# Autodesk Inventor assembly: Electronics
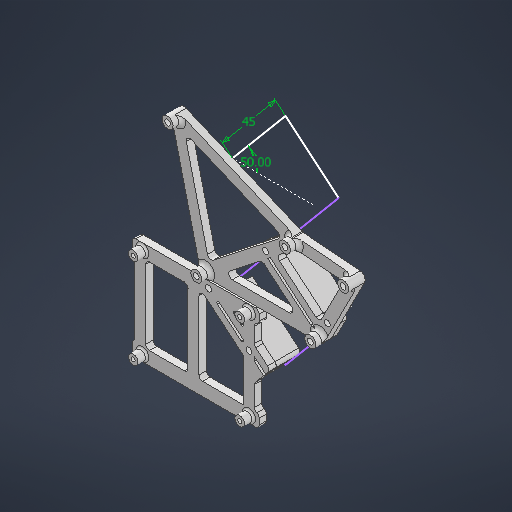
[picture p0: Inventor's stored thumbnail of the model, 512x512]
Saved by Autodesk Inventor 2025 (Build 290162000, 162)
## iProperties
Created: 2024-10-13
Part Number: Electronics
Document SubType Name: Assembly
Designer: Windows 7 was better
Author: Windows 7 was better
## Documents named in this file (6)
- C:\Users\Windows 7 was better\GitHub\ReplicatorPlusConversion\CAD\Inventor\Electronics.iam
- C:\Users\Windows 7 was better\GitHub\ReplicatorPlusConversion\CAD\Inventor\rpi-mount.ipt
- C:\Users\Windows 7 was better\GitHub\ReplicatorPlusConversion\CAD\Inventor\skr-mini-mount.ipt
- C:\Users\Windows 7 was better\GitHub\ReplicatorPlusConversion\STLs\Part1.ipt
- C:\Users\Windows 7 was better\GitHub\ReplicatorPlusConversion\CAD\STEP\rpi-mount-clip.ipt
- C:\Users\Windows 7 was better\GitHub\ReplicatorPlusConversion\CAD\STEP\skr-mini-mount-clip.ipt
## Components (5 placed, 5 different names)
1. rpi-mount:1 — Flush:1
2. skr-mini-mount:1 — Flush:2
3. Part1:1
4. rpi-mount-clip:1 — Flush:1
5. skr-mini-mount-clip:1 — Flush:2
## Relationships (2: Flush 2)
- Flush:1: rpi-mount:1 ↔ rpi-mount-clip:1
- Flush:2: skr-mini-mount:1 ↔ skr-mini-mount-clip:1
